# Autodesk Inventor assembly: Segment_Traeger_v1
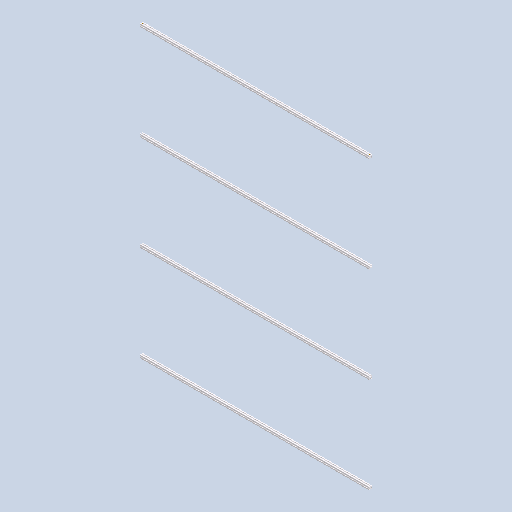
[picture p0: Inventor's stored thumbnail of the model, 512x512]
Saved by Autodesk Inventor 2025.1 (Build 291241000, 241)
## iProperties
Created: 2024-10-13
Part Number: Segment_Traeger_v1
Document SubType Name: Assembly
Designer: Kai Altwicker
Author: Kai Altwicker
## Documents named in this file (3)
- C:\Users\tallA\Repos\VolumanXR\hardware-capture\cad\rig_v1\Segment_Traeger_v1.iam
- C:\Users\tallA\Repos\VolumanXR\hardware-capture\cad\rig_v1\Profil_5_20x20_1500.ipt
- C:\Users\tallA\Repos\VolumanXR\hardware-capture\cad\dimensions.xlsx
## Components (4 placed, 1 different names)
1. Profil_5_20x20_1500:2 — Passend:1, Passend:2
2. Profil_5_20x20_1500:3
3. Profil_5_20x20_1500:4
4. Profil_5_20x20_1500:5
## Component patterns: (4 elements, first: Profil_5_20x20_1500:2)
## Relationships (2: Mate 2)
- Passend:1 [Mate]: Profil_5_20x20_1500:2
- Passend:2 [Mate]: Profil_5_20x20_1500:2
## Named parameters: d_tol = 0.3 mm, d_wand = 1.5 mm, d_traeger = 625 mm, l_profil_40x40 = 2500 mm, h_profil_40x40 = 40 mm, h_profil_20x20 = 20 mm, b_profil_40x40 = 40 mm, b_profil_20x20 = 20 mm, l_profil_20x20 = 1500 mm, D_oct = 3621.32034 mm
